# Autodesk Inventor assembly: Full Chassis Assembly
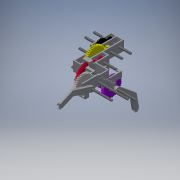
[picture p0: Inventor's stored thumbnail of the model, 180x180]
Saved by Autodesk Inventor 2017 (Build 210142000, 142)
## iProperties
Created: 2019-12-02
Part Number: Full Chassis Assembly
Document SubType Name: Assembly
Designer: asadb
Author: asadb
## Documents named in this file (11)
- C:\Users\asadb\Desktop\University\Courses\Engineering 1C03 - Eng Design and Graphics\Asad Chassis\Full Chassis Assembly.iam
- C:\Users\asadb\Desktop\University\Courses\Engineering 1C03 - Eng Design and Graphics\Asad Chassis\Gear Train Chassis Version 2.ipt
- C:\Users\asadb\Desktop\University\Courses\Engineering 1C03 - Eng Design and Graphics\Asad Chassis\Spur Gear (12mm).ipt
- C:\Users\asadb\Desktop\University\Courses\Engineering 1C03 - Eng Design and Graphics\Asad Chassis\Spur Gear (24mm).ipt
- C:\Users\asadb\Desktop\University\Courses\Engineering 1C03 - Eng Design and Graphics\Asad Chassis\3in rod.ipt
- C:\Users\asadb\Desktop\University\Courses\Engineering 1C03 - Eng Design and Graphics\Asad Chassis\Spur Gear (39mm).ipt
- C:\Users\asadb\Desktop\University\Courses\Engineering 1C03 - Eng Design and Graphics\Asad Chassis\Spur Gear (48mm).ipt
- C:\Users\asadb\Desktop\University\Courses\Engineering 1C03 - Eng Design and Graphics\Asad Chassis\Spur Gear (36mm).ipt
- C:\Users\asadb\Desktop\University\Courses\Engineering 1C03 - Eng Design and Graphics\Asad Chassis\Spur Gear (13mm).ipt
- C:\Users\asadb\Desktop\University\Courses\Engineering 1C03 - Eng Design and Graphics\Asad Chassis\Finger.ipt
- C:\Users\asadb\Desktop\University\Courses\Engineering 1C03 - Eng Design and Graphics\Asad Chassis\Finger (Index).ipt
## Components (21 placed, 6 different names)
1. Gear Train Chassis Version 2:1 — Rotational:1, Rotational:2, Rotational:3, Rotational:4, Rotational:5, Rigid:7, Rotational:6
2. Spur Gear1:1 — Mate:1, Rigid:2, Rotation:1
3. Spur Gear2:1 — Rigid:1, Rotation:1
4. 3in rod:1 — Rotational:1, Mate:1, Rigid:2
5. 3in rod:2 — Rigid:1, Rotational:2, Mate:2, Rigid:3
6. 3in rod:3 — Rotational:3, Mate:3, Rigid:4, Mate:4, Rigid:5
7. Spur Gear1:2 — Mate:2, Rigid:3, Rotation:2
8. Spur Gear1:3 — Mate:4, Rigid:5, Rotation:3
9. Spur Gear1:4 — Mate:3, Rigid:4, Rotation:2
10. 3in rod:4 — Rotational:4, Mate:5, Rigid:6, Mate:6, Rigid:8, Rigid:10
11. Spur Gear2:2 — Mate:5, Rigid:6, Rotation:3
12. 3in rod:5 — Rotational:6, Mate:7, Rigid:9, Mate:12, Flush:2
13. 3in rod:6 — Rigid:7, Rotational:7
14. 3in rod:7 — Rotational:5, Mate:9, Rigid:11, Mate:10, Flush:1, Angle:15
15. Spur Gear1:5 — Mate:6, Rigid:8, Rotation:4
16. Spur Gear1:6 — Rigid:10, Rotation:5
17. Spur Gear1:7 — Mate:9, Rigid:11, Rotation:6
18. Spur Gear1:8 — Mate:7, Rigid:9, Rotation:4, Flush:14
19. Spur Gear1:9 — Rotational:7, Rotation:5, Rotation:6
20. Finger:1 — Mate:12, Flush:2, Flush:14
21. Finger (Index):1 — Mate:10, Flush:1, Angle:15
## Relationships (38: WeldJoint 11, Mate 10, RevoluteJoint 7, RelateRotation 6, Flush 3, Angle 1)
- Rotational:1 [RevoluteJoint]: Gear Train Chassis Version 2:1 ↔ 3in rod:1
- Mate:1: Spur Gear1:1 ↔ 3in rod:1
- Rigid:1 [WeldJoint] (-30.075 mm): Spur Gear2:1 ↔ 3in rod:2
- Rotational:2 [RevoluteJoint]: Gear Train Chassis Version 2:1 ↔ 3in rod:2
- Rigid:2 [WeldJoint] (-30.075 mm): Spur Gear1:1 ↔ 3in rod:1
- Rotation:1 [RelateRotation] (0.5 ul): Spur Gear1:1 ↔ Spur Gear2:1
- Rotational:3 [RevoluteJoint]: Gear Train Chassis Version 2:1 ↔ 3in rod:3
- Mate:2: 3in rod:2 ↔ Spur Gear1:2
- Rigid:3 [WeldJoint] (-28.975 mm): 3in rod:2 ↔ Spur Gear1:2
- Mate:3: 3in rod:3 ↔ Spur Gear1:4
- Rigid:4 [WeldJoint] (-28.975 mm): 3in rod:3 ↔ Spur Gear1:4
- Rotation:2 [RelateRotation] (0.3077 ul): Spur Gear1:2 ↔ Spur Gear1:4
- Mate:4: 3in rod:3 ↔ Spur Gear1:3
- Rigid:5 [WeldJoint] (-29.586 mm): 3in rod:3 ↔ Spur Gear1:3
- Rotational:4 [RevoluteJoint]: Gear Train Chassis Version 2:1 ↔ 3in rod:4
- Mate:5: 3in rod:4 ↔ Spur Gear2:2
- Rigid:6 [WeldJoint] (-29.586 mm): 3in rod:4 ↔ Spur Gear2:2
- Rotation:3 [RelateRotation] (0.25 ul): Spur Gear1:3 ↔ Spur Gear2:2
- Rotational:5 [RevoluteJoint] (-12 mm): Gear Train Chassis Version 2:1 ↔ 3in rod:7
- Rigid:7 [WeldJoint]: Gear Train Chassis Version 2:1 ↔ 3in rod:6
- Rotational:6 [RevoluteJoint]: Gear Train Chassis Version 2:1 ↔ 3in rod:5
- Mate:6: 3in rod:4 ↔ Spur Gear1:5
- Rigid:8 [WeldJoint] (-13.029 mm): 3in rod:4 ↔ Spur Gear1:5
- Mate:7: 3in rod:5 ↔ Spur Gear1:8
- Rigid:9 [WeldJoint] (-50.029 mm): 3in rod:5 ↔ Spur Gear1:8
- Rotation:4 [RelateRotation] (0.3333 ul): Spur Gear1:5 ↔ Spur Gear1:8
- Rigid:10 [WeldJoint] (-18.025 mm): 3in rod:4 ↔ Spur Gear1:6
- Rotational:7 [RevoluteJoint] (-65.908 mm): 3in rod:6 ↔ Spur Gear1:9
- Rotation:5 [RelateRotation] (0.9231 ul): Spur Gear1:6 ↔ Spur Gear1:9
- Mate:9: 3in rod:7 ↔ Spur Gear1:7
- Rigid:11 [WeldJoint] (-57 mm): 3in rod:7 ↔ Spur Gear1:7
- Rotation:6 [RelateRotation] (0.3611 ul): Spur Gear1:7 ↔ Spur Gear1:9
- Mate:10: 3in rod:7 ↔ Finger (Index):1
- Flush:1 (40 mm): 3in rod:7 ↔ Finger (Index):1
- Mate:12: 3in rod:5 ↔ Finger:1
- Flush:2 (38 mm): 3in rod:5 ↔ Finger:1
- Flush:14: Spur Gear1:8 ↔ Finger:1
- Angle:15 (140 deg): 3in rod:7 ↔ Finger (Index):1
